# Autodesk Inventor assembly: Ensamblaje_tapa_inferior_mesa
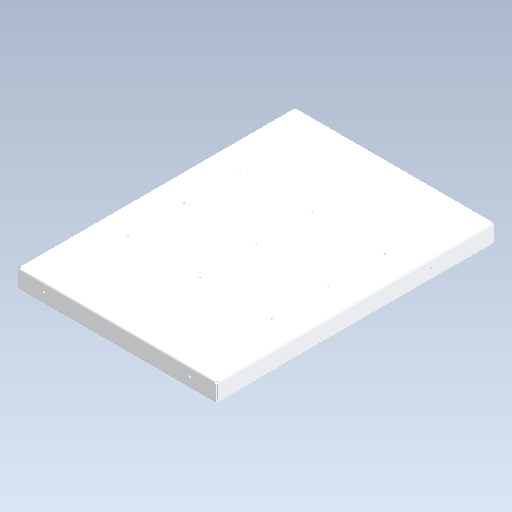
[picture p0: Inventor's stored thumbnail of the model, 512x512]
Saved by Autodesk Inventor 2021 (Build 250183000, 183)
## iProperties
Created: 2021-05-06
Part Number: Ensamblaje_tapa_inferior_mesa
Document SubType Name: Assembly
Designer: Admin
Author: Admin
## Documents named in this file (3)
- D:\Nelson\Documentos\Inventor\Proyecto_PAI\Ensamblaje_tapa_inferior_mesa.iam
- D:\Nelson\Documentos\Inventor\Proyecto_PAI\TapaBMesa.ipt
- D:\Nelson\Documentos\Inventor\Proyecto_PAI\Base_Ruedas.ipt
## Components (5 placed, 2 different names)
1. TapaBMesa:1 — Coincidencia:1, Coincidencia:2, Coincidencia:3, Coincidencia:4, Coincidencia:5, Coincidencia:6, Coincidencia:7, Coincidencia:8, Coincidencia:9, Coincidencia:11, Coincidencia:12
2. Base_Ruedas:1 — Coincidencia:7, Coincidencia:8, Coincidencia:9
3. Base_Ruedas:2 — Coincidencia:1, Coincidencia:2, Coincidencia:3
4. Base_Ruedas:3 — Coincidencia:4, Coincidencia:5, Coincidencia:6
5. Base_Ruedas:4 — Coincidencia:11, Coincidencia:12
## Relationships (11: Mate 11)
- Coincidencia:1 [Mate]: TapaBMesa:1 ↔ Base_Ruedas:2
- Coincidencia:2 [Mate]: TapaBMesa:1 ↔ Base_Ruedas:2
- Coincidencia:3 [Mate]: TapaBMesa:1 ↔ Base_Ruedas:2
- Coincidencia:4 [Mate]: TapaBMesa:1 ↔ Base_Ruedas:3
- Coincidencia:5 [Mate]: TapaBMesa:1 ↔ Base_Ruedas:3
- Coincidencia:6 [Mate]: TapaBMesa:1 ↔ Base_Ruedas:3
- Coincidencia:7 [Mate]: TapaBMesa:1 ↔ Base_Ruedas:1
- Coincidencia:8 [Mate]: TapaBMesa:1 ↔ Base_Ruedas:1
- Coincidencia:9 [Mate]: TapaBMesa:1 ↔ Base_Ruedas:1
- Coincidencia:11 [Mate]: TapaBMesa:1 ↔ Base_Ruedas:4
- Coincidencia:12 [Mate]: TapaBMesa:1 ↔ Base_Ruedas:4
